# Autodesk Inventor assembly: Gruppe
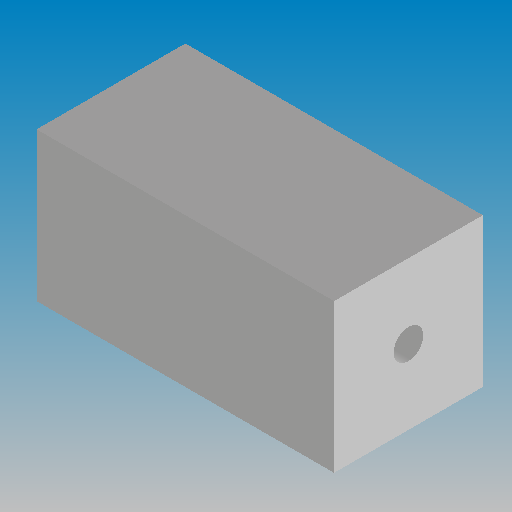
[picture p0: Inventor's stored thumbnail of the model, 512x512]
Saved by Autodesk Inventor 2021 (Build 250183000, 183)
## iProperties
Created: 2021-08-27
Part Number: Gruppe
Document SubType Name: Assembly
Designer: Rama
Author: Rama
## Documents named in this file (3)
- C:\Users\Rama\Desktop\GitHub\Voron-2-Mods\Misumi_RBPB5\CAD\Src\Z-Joint_Base.iam
- C:\Users\Rama\Desktop\GitHub\Voron-2-Mods\Misumi_RBPB5\CAD\Src\Z-Joint_Base.ipt
- C:\Users\Rama\Desktop\GitHub\Voron-2-Mods\Misumi_RBPB5\CAD\Src\RBPB5-Bearing\RBPB5.iam
## Components (2 placed, 2 different names)
1. Z-Joint:1 — Passend:2, Fluchtend:1
2. RBPB5:1 [sub-assembly] — Passend:2, Fluchtend:1
## Relationships (2: Mate 1, Flush 1)
- Passend:2 [Mate]: Z-Joint:1 ↔ RBPB5:1
- Fluchtend:1 [Flush]: Z-Joint:1 ↔ RBPB5:1
